# Autodesk Inventor assembly: Assembly Rev C
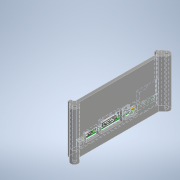
[picture p0: Inventor's stored thumbnail of the model, 180x180]
Saved by Autodesk Inventor 2021 (Build 250183000, 183)
## iProperties
Created: 2021-07-26
Part Number: Assembly Rev C
Document SubType Name: Assembly
Designer: cmzgt
Author: cmzgt
## Documents named in this file (3)
- D:\Projects\3D Designs\RPICase\Rev C\Assembly Rev C.iam
- D:\Projects\3D Designs\RPICase\Rev C\Case RevC.ipt
- C:\Users\cmzgt\Desktop\RPi Model\Raspberry Pi 3.iam
## Components (2 placed, 2 different names)
1. Case RevC:1 — Mate:1, Mate:2
2. Raspberry Pi 3:1 [sub-assembly] — Mate:1, Mate:2
## Relationships (2: Mate 2)
- Mate:1: Case RevC:1 ↔ Raspberry Pi 3:1
- Mate:2: Case RevC:1 ↔ Raspberry Pi 3:1
